# Autodesk Inventor assembly: LeftMecanum-SubAssem01
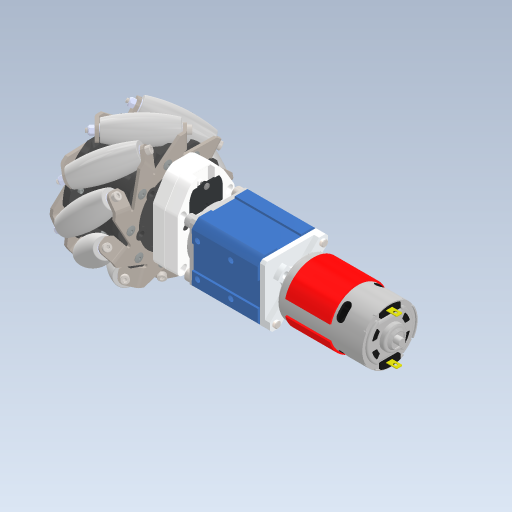
[picture p0: Inventor's stored thumbnail of the model, 512x512]
Saved by Autodesk Inventor 2023 (Build 270158000, 158)
## iProperties
Created: 2022-07-11
Part Number: LeftMecanum-SubAssem01
Document SubType Name: Assembly
Designer: Dave
Author: Dave
## Documents named in this file (6)
- C:\Users\Dave\Documents\GrabCAD\Chalk Bot\Chalkbot1.0\Chassis\V1\LeftMecanum-SubAssem01.iam
- C:\Users\Dave\Documents\GrabCAD\Chalk Bot\Chalkbot1.0\Chassis\V1\Mechanum STEP files\am-3775a AndyMark RedLine Motor (1).ipt
- C:\Users\Dave\Documents\GrabCAD\Chalk Bot\Chalkbot1.0\Chassis\V1\Motor and Gearbox STEP files\Hex Bore Mag Encoder Housing (217-6785).iam
- C:\Users\Dave\Documents\GrabCAD\Chalk Bot\Chalkbot1.0\Chassis\V1\Motor and Gearbox STEP files\am-3791 - 3000 x 500 Hex Shaft.ipt
- C:\Users\Dave\Documents\GrabCAD\Chalk Bot\Chalkbot1.0\Chassis\V1\Motor and Gearbox STEP files\2 Stage HD - 57 Sport.ipt
- C:\Users\Dave\Documents\GrabCAD\Chalk Bot\Chalkbot1.0\Chassis\V1\Mechanum STEP files\am-3918R 4HD 500H Mecanum Left.iam
## Components (5 placed, 5 different names)
1. 2 Stage HD - 57 Sport:1 — Insert:4, Insert:5, Angle:1, Mate:10
2. am-3775a AndyMark RedLine Motor (1):1 — Mate:9, Insert:5
3. Hex Bore Mag Encoder Housing (217-6785):1 [sub-assembly] — Mate:9, Mate:10
4. am-3791 - 3000 x 500 Hex Shaft:1 — Insert:4, Mate:11, Mate:12, Flush:1
5. am-3918R 4HD 500H Mecanum Left:1 [sub-assembly] — Mate:11, Mate:12, Flush:1
## Relationships (11: Insert 5, Mate 4, Angle 1, Flush 1)
- [Insert]: 2 Stage HD - 57 Sport:1 ↔ am-3775a AndyMark RedLine Motor (1):1
- [Insert]: 2 Stage HD - 57 Sport:1 ↔ am-3775a AndyMark RedLine Motor (1):1
- [Insert]: 2 Stage HD - 57 Sport:1 ↔ am-3791 - 3000 x 500 Hex Shaft:1
- Insert:4: 2 Stage HD - 57 Sport:1 ↔ am-3791 - 3000 x 500 Hex Shaft:1
- Mate:9: am-3775a AndyMark RedLine Motor (1):1 ↔ Hex Bore Mag Encoder Housing (217-6785):1
- Insert:5: 2 Stage HD - 57 Sport:1 ↔ am-3775a AndyMark RedLine Motor (1):1
- Angle:1 (0 deg): 2 Stage HD - 57 Sport:1
- Mate:10: 2 Stage HD - 57 Sport:1 ↔ Hex Bore Mag Encoder Housing (217-6785):1
- Mate:11: am-3791 - 3000 x 500 Hex Shaft:1 ↔ am-3918R 4HD 500H Mecanum Left:1
- Mate:12: am-3791 - 3000 x 500 Hex Shaft:1 ↔ am-3918R 4HD 500H Mecanum Left:1
- Flush:1: am-3791 - 3000 x 500 Hex Shaft:1 ↔ am-3918R 4HD 500H Mecanum Left:1
